# Autodesk Inventor assembly: modularRICHTurntable
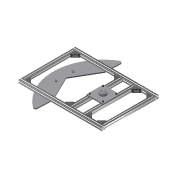
[picture p0: Inventor's stored thumbnail of the model, 180x180]
Saved by Autodesk Inventor 2018.2 (Build 222227000, 227)
## iProperties
Created: 2018-05-06
Part Number: modularRICHTurntable
Document SubType Name: Assembly
Designer: sawaiz
Author: sawaiz
## Documents named in this file (13)
- C:\Users\sawaiz\OneDrive\projects\modularRICHTurntable\modularRICHTurntable.iam
- C:\Users\sawaiz\OneDrive\projects\modularRICHTurntable\frame\hfs5-2020Depth.ipt
- C:\Users\sawaiz\OneDrive\projects\modularRICHTurntable\frame\hfs5-2020Width.ipt
- C:\Users\sawaiz\OneDrive\projects\modularRICHTurntable\hardware\angleBracket.iam
- C:\Users\sawaiz\Desktop\5909K330_THRUST NEEDLE-ROLLER BEARING.ipt
- C:\Users\sawaiz\Desktop\5909K590_THRUST NEEDLE-ROLLER BEARING.ipt
- C:\Users\sawaiz\Desktop\6435K160_ONE-PIECE CLAMP-ON SHAFT COLLAR.ipt
- C:\Users\sawaiz\Desktop\2025K180_303 SS SHAFT WITH RETAINING RING GROOVES.ipt
- C:\Users\sawaiz\OneDrive\projects\modularRICHTurntable\topPlate.ipt
- C:\Users\sawaiz\OneDrive\projects\modularRICHTurntable\hardware\m5TNut.ipt
- C:\Users\sawaiz\OneDrive\projects\modularRICHTurntable\hardware\m5x12BlackSocketHead.ipt
- C:\Users\sawaiz\Desktop\94669A168_ALUM UNTHRD SPACER.ipt
- C:\Users\sawaiz\OneDrive\projects\modularRICHTurntable\beltMount.ipt
## Components (35 placed, 12 different names)
1. hfs5-2020Depth:1 — Flush:1, Flush:2, Symmetry:1, Symmetry:2, Symmetry:3, Mate:3, Mate:4, Mate:6, Flush:8, Mate:42, Mate:43, Mate:49
2. hfs5-2020Depth:2 — Flush:1, Flush:2, Symmetry:1, Symmetry:2, Symmetry:3, Mate:1, Mate:2, Flush:3, Flush:4, Flush:5, Flush:6, Mate:5, Mate:7, Flush:7, Flush:11, Flush:12, Mate:16, Mate:40, Mate:41, Mate:44
3. hfs5-2020Width:1 — Mate:1, Flush:4, Flush:5, Mate:8, Mate:9
4. hfs5-2020Width:2 — Mate:2, Flush:3, Flush:6, Mate:3, Mate:10, Mate:11, Flush:9, Flush:10
5. angleBracket:1 [sub-assembly] — Mate:7, Mate:9, Flush:7
6. angleBracket:2 [sub-assembly] — Mate:6, Mate:8, Flush:8
7. angleBracket:3 [sub-assembly] — Mate:4, Mate:10, Flush:10
8. angleBracket:4 [sub-assembly] — Mate:5, Mate:11, Flush:9
9. hfs5-2020Width:3 — Flush:11, Flush:13, Mate:18, Flush:15, Angle:2, Mate:37, Mate:38, Flush:23, Flush:24
10. hfs5-2020Width:4 — Flush:12, Flush:13, Mate:16, Flush:14, Mate:36, Mate:39, Flush:22, Flush:25
11. 5909K330_THRUST NEEDLE-ROLLER BEARING:1 — Tangent:1, Tangent:2, Mate:12, Tangent:3
12. 5909K590_THRUST NEEDLE-ROLLER BEARING:1 — Tangent:1, Tangent:2, Mate:13, Mate:21
13. 6435K160_ONE-PIECE CLAMP-ON SHAFT COLLAR:1 — Mate:15, Mate:17, Mate:21
14. 5909K590_THRUST NEEDLE-ROLLER BEARING:2 — Mate:12, Mate:13, Tangent:3, Mate:14, Mate:20
15. 6435K160_ONE-PIECE CLAMP-ON SHAFT COLLAR:2 — Mate:14, Mate:15, Flush:16, Mate:22
16. 2025K180_303 SS SHAFT WITH RETAINING RING GROOVES:1 — Mate:17, Mate:19, Flush:16, Mate:54
17. topPlate:1 — Mate:18, Flush:14, Flush:15, Mate:19, Mate:20, Mate:22, Mate:31, Mate:32, Mate:33, Mate:34, Mate:35
18. m5TNut:1 — Mate:23, Mate:24, Flush:20, Angle:1, Symmetry:4
19. m5x12BlackSocketHead:1 — Mate:23, Mate:24, Mate:34, Flush:19
20. m5TNut:2 — Flush:21
21. m5x12BlackSocketHead:2 — Mate:31, Flush:17, Mate:35
22. m5TNut:3 — Flush:21, Angle:1, Angle:2
23. m5x12BlackSocketHead:3 — Mate:33, Flush:17, Flush:18
24. m5TNut:4 — Flush:20, Symmetry:4
25. m5x12BlackSocketHead:4 — Mate:32, Flush:18, Flush:19
26. angleBracket:5 [sub-assembly] — Mate:39, Mate:41, Flush:25
27. angleBracket:6 [sub-assembly] — Mate:36, Mate:43, Flush:22
28. angleBracket:7 [sub-assembly] — Mate:37, Mate:42, Flush:23
29. angleBracket:8 [sub-assembly] — Mate:38, Mate:40, Flush:24
30. 94669A168_ALUM UNTHRD SPACER:1 — Mate:44, Mate:45, Flush:27, Mate:52
31. beltMount:1 — Mate:46, Flush:26, Mate:47, Mate:52, Mate:53
32. beltMount:2 — Mate:45, Mate:46, Flush:26, Mate:47, Mate:48, Mate:50, Mate:51, Mate:54
33. 94669A168_ALUM UNTHRD SPACER:2 — Flush:27, Flush:28, Mate:53
34. 94669A168_ALUM UNTHRD SPACER:3 — Flush:28, Flush:29, Mate:48, Mate:49, Mate:50
35. 94669A168_ALUM UNTHRD SPACER:4 — Flush:29, Mate:51
## Relationships (92: Mate 54, Flush 29, Symmetry 4, Tangent 3, Angle 2)
- Flush:1: hfs5-2020Depth:1 ↔ hfs5-2020Depth:2
- Flush:2: hfs5-2020Depth:1 ↔ hfs5-2020Depth:2
- Symmetry:1: hfs5-2020Depth:1 ↔ hfs5-2020Depth:2
- Symmetry:2: hfs5-2020Depth:1 ↔ hfs5-2020Depth:2
- Symmetry:3: hfs5-2020Depth:1 ↔ hfs5-2020Depth:2
- Mate:1: hfs5-2020Depth:2 ↔ hfs5-2020Width:1
- Mate:2: hfs5-2020Depth:2 ↔ hfs5-2020Width:2
- Flush:3: hfs5-2020Depth:2 ↔ hfs5-2020Width:2
- Flush:4: hfs5-2020Depth:2 ↔ hfs5-2020Width:1
- Flush:5: hfs5-2020Depth:2 ↔ hfs5-2020Width:1
- Flush:6: hfs5-2020Depth:2 ↔ hfs5-2020Width:2
- Mate:3: hfs5-2020Depth:1 ↔ hfs5-2020Width:2
- Mate:4: hfs5-2020Depth:1 ↔ angleBracket:3
- Mate:5: hfs5-2020Depth:2 ↔ angleBracket:4
- Mate:6: hfs5-2020Depth:1 ↔ angleBracket:2
- Mate:7: hfs5-2020Depth:2 ↔ angleBracket:1
- Mate:8: hfs5-2020Width:1 ↔ angleBracket:2
- Mate:9: hfs5-2020Width:1 ↔ angleBracket:1
- Flush:7: hfs5-2020Depth:2 ↔ angleBracket:1
- Flush:8: hfs5-2020Depth:1 ↔ angleBracket:2
- Mate:10: hfs5-2020Width:2 ↔ angleBracket:3
- Mate:11: hfs5-2020Width:2 ↔ angleBracket:4
- Flush:9: hfs5-2020Width:2 ↔ angleBracket:4
- Flush:10: hfs5-2020Width:2 ↔ angleBracket:3
- Tangent:1: 5909K330_THRUST NEEDLE-ROLLER BEARING:1 ↔ 5909K590_THRUST NEEDLE-ROLLER BEARING:1
- Tangent:2: 5909K330_THRUST NEEDLE-ROLLER BEARING:1 ↔ 5909K590_THRUST NEEDLE-ROLLER BEARING:1
- Mate:12: 5909K330_THRUST NEEDLE-ROLLER BEARING:1 ↔ 5909K590_THRUST NEEDLE-ROLLER BEARING:2
- Mate:13: 5909K590_THRUST NEEDLE-ROLLER BEARING:1 ↔ 5909K590_THRUST NEEDLE-ROLLER BEARING:2
- Tangent:3: 5909K330_THRUST NEEDLE-ROLLER BEARING:1 ↔ 5909K590_THRUST NEEDLE-ROLLER BEARING:2
- Mate:14: 5909K590_THRUST NEEDLE-ROLLER BEARING:2 ↔ 6435K160_ONE-PIECE CLAMP-ON SHAFT COLLAR:2
- Mate:15: 6435K160_ONE-PIECE CLAMP-ON SHAFT COLLAR:1 ↔ 6435K160_ONE-PIECE CLAMP-ON SHAFT COLLAR:2
- Flush:11: hfs5-2020Depth:2 ↔ hfs5-2020Width:3
- Flush:12: hfs5-2020Depth:2 ↔ hfs5-2020Width:4
- Flush:13: hfs5-2020Width:3 ↔ hfs5-2020Width:4
- Mate:16: hfs5-2020Depth:2 ↔ hfs5-2020Width:4
- Mate:17: 6435K160_ONE-PIECE CLAMP-ON SHAFT COLLAR:1 ↔ 2025K180_303 SS SHAFT WITH RETAINING RING GROOVES:1
- Mate:18: hfs5-2020Width:3 ↔ topPlate:1
- Flush:14: hfs5-2020Width:4 ↔ topPlate:1
- Flush:15: hfs5-2020Width:3 ↔ topPlate:1
- Mate:19: 2025K180_303 SS SHAFT WITH RETAINING RING GROOVES:1 ↔ topPlate:1
- Mate:20: 5909K590_THRUST NEEDLE-ROLLER BEARING:2 ↔ topPlate:1
- Mate:21: 5909K590_THRUST NEEDLE-ROLLER BEARING:1 ↔ 6435K160_ONE-PIECE CLAMP-ON SHAFT COLLAR:1
- Flush:16: 6435K160_ONE-PIECE CLAMP-ON SHAFT COLLAR:2 ↔ 2025K180_303 SS SHAFT WITH RETAINING RING GROOVES:1
- Mate:22: 6435K160_ONE-PIECE CLAMP-ON SHAFT COLLAR:2 ↔ topPlate:1
- Mate:23: m5TNut:1 ↔ m5x12BlackSocketHead:1
- Mate:24 (8.35 mm): m5TNut:1 ↔ m5x12BlackSocketHead:1
- [Mate]: m5TNut:2 ↔ m5x12BlackSocketHead:2
- [Mate] (8.35 mm): m5TNut:2 ↔ m5x12BlackSocketHead:2
- [Mate]: m5TNut:3 ↔ m5x12BlackSocketHead:3
- [Mate] (8.35 mm): m5TNut:3 ↔ m5x12BlackSocketHead:3
- [Mate]: m5TNut:4 ↔ m5x12BlackSocketHead:4
- [Mate] (8.35 mm): m5TNut:4 ↔ m5x12BlackSocketHead:4
- Mate:31: topPlate:1 ↔ m5x12BlackSocketHead:2
- Mate:32: topPlate:1 ↔ m5x12BlackSocketHead:4
- Mate:33: topPlate:1 ↔ m5x12BlackSocketHead:3
- Mate:34: topPlate:1 ↔ m5x12BlackSocketHead:1
- Flush:17: m5x12BlackSocketHead:2 ↔ m5x12BlackSocketHead:3
- Flush:18: m5x12BlackSocketHead:3 ↔ m5x12BlackSocketHead:4
- Flush:19: m5x12BlackSocketHead:1 ↔ m5x12BlackSocketHead:4
- Flush:20: m5TNut:1 ↔ m5TNut:4
- Flush:21: m5TNut:2 ↔ m5TNut:3
- Angle:1 (0 deg): m5TNut:1 ↔ m5TNut:3
- Angle:2 (0 deg): hfs5-2020Width:3 ↔ m5TNut:3
- Mate:35: topPlate:1 ↔ m5x12BlackSocketHead:2
- Mate:36: hfs5-2020Width:4 ↔ angleBracket:6
- Mate:37: hfs5-2020Width:3 ↔ angleBracket:7
- Mate:38: hfs5-2020Width:3 ↔ angleBracket:8
- Mate:39: hfs5-2020Width:4 ↔ angleBracket:5
- Mate:40: hfs5-2020Depth:2 ↔ angleBracket:8
- Mate:41: hfs5-2020Depth:2 ↔ angleBracket:5
- Mate:42: hfs5-2020Depth:1 ↔ angleBracket:7
- Mate:43: hfs5-2020Depth:1 ↔ angleBracket:6
- Flush:22: hfs5-2020Width:4 ↔ angleBracket:6
- Flush:23: hfs5-2020Width:3 ↔ angleBracket:7
- Flush:24: hfs5-2020Width:3 ↔ angleBracket:8
- Flush:25: hfs5-2020Width:4 ↔ angleBracket:5
- Symmetry:4: m5TNut:1 ↔ m5TNut:4
- Mate:44: hfs5-2020Depth:2 ↔ 94669A168_ALUM UNTHRD SPACER:1
- Mate:45: 94669A168_ALUM UNTHRD SPACER:1 ↔ beltMount:2
- Mate:46: beltMount:1 ↔ beltMount:2
- Flush:26: beltMount:1 ↔ beltMount:2
- Mate:47: beltMount:1 ↔ beltMount:2
- Flush:27: 94669A168_ALUM UNTHRD SPACER:1 ↔ 94669A168_ALUM UNTHRD SPACER:2
- Flush:28: 94669A168_ALUM UNTHRD SPACER:2 ↔ 94669A168_ALUM UNTHRD SPACER:3
- Flush:29: 94669A168_ALUM UNTHRD SPACER:3 ↔ 94669A168_ALUM UNTHRD SPACER:4
- Mate:48: beltMount:2 ↔ 94669A168_ALUM UNTHRD SPACER:3
- Mate:49: hfs5-2020Depth:1 ↔ 94669A168_ALUM UNTHRD SPACER:3
- Mate:50: beltMount:2 ↔ 94669A168_ALUM UNTHRD SPACER:3
- Mate:51: beltMount:2 ↔ 94669A168_ALUM UNTHRD SPACER:4
- Mate:52: 94669A168_ALUM UNTHRD SPACER:1 ↔ beltMount:1
- Mate:53: beltMount:1 ↔ 94669A168_ALUM UNTHRD SPACER:2
- Mate:54: 2025K180_303 SS SHAFT WITH RETAINING RING GROOVES:1 ↔ beltMount:2
## Named parameters: d45_d43 = 0 mm, d46_d44 = 8.35 mm, d47_d43 = 0 mm, d48_d44 = 8.35 mm, d49_d43 = 0 mm, d50_d44 = 8.35 mm
